# Autodesk Inventor assembly: boardB
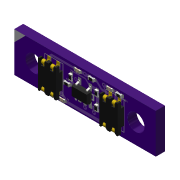
[picture p0: Inventor's stored thumbnail of the model, 180x180]
Saved by Autodesk Inventor 2017 (Build 210142000, 142)
## iProperties
Created: 2016-02-15
Part Number: boardB
Document SubType Name: Assembly
Designer: sawai
Author: sawai
## Documents named in this file (11)
- C:\Users\sawaiz\oneDrive\projects\mppcSensor\cad\sensorBoardB\boardB.iam
- C:\Users\sawaiz\oneDrive\projects\mppcSensor\cad\electronics\788640001\788640001.iam
- C:\Users\sawaiz\OneDrive\projects\mppcSensor\cad\electronics\chipResistor.ipt
- C:\Users\sawaiz\oneDrive\projects\mppcSensor\cad\sensorBoardB\boardB.ipt
- C:\Users\sawaiz\oneDrive\projects\mppcSensor\cad\electronics\SOT23-5.ipt
- C:\Users\sawaiz\oneDrive\projects\mppcSensor\cad\electronics\chipResistor\chipResistor-0402.ipt
- C:\Users\sawaiz\oneDrive\projects\mppcSensor\cad\electronics\capacitor\capacitor-0402.ipt
- C:\Users\sawaiz\oneDrive\projects\mppcSensor\cad\electronics\capacitor.ipt
- C:\Users\sawaiz\oneDrive\projects\mppcSensor\cad\electronics\LTST-S270GKT.ipt
- C:\Users\sawaiz\oneDrive\projects\mppcSensor\cad\electronics\chipResistor\chipResistor-0603.ipt
- C:\Users\sawaiz\oneDrive\projects\mppcSensor\cad\electronics\13360-20xx-VE\13360-30xxVE.ipt
## Components (17 placed, 8 different names)
1. 788640001:1 [sub-assembly] — Flush:1, Angle:2, Mate:1
2. 788640001:2 [sub-assembly] — Flush:1, Angle:2
3. boardB:1 — Mate:1, Mate:2, Angle:3, Angle:4, Mate:3, Angle:13, Mate:4, Mate:5, Angle:14, Angle:15, Angle:16
4. SOT23-5:1 — Mate:2, Angle:3
5. chipResistor-0402:1 — Flush:2, Angle:10
6. chipResistor-0402:2 — Flush:2, Flush:3, Angle:9, Angle:10
7. chipResistor-0402:3 — Flush:3, Flush:4, Angle:8, Angle:9
8. chipResistor-0402:4 — Flush:4, Flush:5, Angle:6, Angle:7
9. chipResistor-0402:5 — Flush:6, Flush:7, Angle:5, Angle:6
10. chipResistor-0402:6 — Flush:5, Flush:6, Angle:7, Angle:8, Mate:3
11. chipResistor-0402:7 — Flush:7, Angle:4, Angle:5
12. capacitor-0402:1 — Flush:9, Angle:12, Angle:13
13. capacitor-0402:2 — Flush:8, Flush:9, Angle:11, Angle:12
14. capacitor-0402:3 — Flush:8, Angle:11, Mate:4
15. LTST-S270GKT:1 — Flush:10, Flush:11, Angle:16
16. chipResistor-0603:8 — Flush:10, Angle:15
17. 13360-30xxVE:1 — Flush:11, Mate:5, Angle:14
## Relationships (31: Angle 15, Flush 11, Mate 5)
- Flush:1: 788640001:1 ↔ 788640001:2
- Angle:2 (0 deg): 788640001:1 ↔ 788640001:2
- Mate:1: 788640001:1 ↔ boardB:1
- Mate:2: boardB:1 ↔ SOT23-5:1
- Angle:3 (0 deg): boardB:1 ↔ SOT23-5:1
- Flush:2: chipResistor-0402:1 ↔ chipResistor-0402:2
- Flush:3: chipResistor-0402:2 ↔ chipResistor-0402:3
- Flush:4: chipResistor-0402:3 ↔ chipResistor-0402:4
- Flush:5: chipResistor-0402:4 ↔ chipResistor-0402:6
- Flush:6: chipResistor-0402:5 ↔ chipResistor-0402:6
- Flush:7: chipResistor-0402:5 ↔ chipResistor-0402:7
- Angle:4 (0 deg): boardB:1 ↔ chipResistor-0402:7
- Angle:5 (0 deg): chipResistor-0402:5 ↔ chipResistor-0402:7
- Angle:6 (0 deg): chipResistor-0402:4 ↔ chipResistor-0402:5
- Angle:7 (0 deg): chipResistor-0402:4 ↔ chipResistor-0402:6
- Angle:8 (0 deg): chipResistor-0402:3 ↔ chipResistor-0402:6
- Angle:9 (0 deg): chipResistor-0402:2 ↔ chipResistor-0402:3
- Angle:10 (0 deg): chipResistor-0402:1 ↔ chipResistor-0402:2
- Mate:3: boardB:1 ↔ chipResistor-0402:6
- Flush:8: capacitor-0402:2 ↔ capacitor-0402:3
- Flush:9: capacitor-0402:1 ↔ capacitor-0402:2
- Angle:11 (0 deg): capacitor-0402:2 ↔ capacitor-0402:3
- Angle:12 (0 deg): capacitor-0402:1 ↔ capacitor-0402:2
- Angle:13 (0 deg): boardB:1 ↔ capacitor-0402:1
- Mate:4: boardB:1 ↔ capacitor-0402:3
- Flush:10: LTST-S270GKT:1 ↔ chipResistor-0603:8
- Flush:11: LTST-S270GKT:1 ↔ 13360-30xxVE:1
- Mate:5: boardB:1 ↔ 13360-30xxVE:1
- Angle:14 (45 deg): boardB:1 ↔ 13360-30xxVE:1
- Angle:15 (0 deg): boardB:1 ↔ chipResistor-0603:8
- Angle:16 (0 deg): boardB:1 ↔ LTST-S270GKT:1
